# Autodesk Inventor assembly: playwood
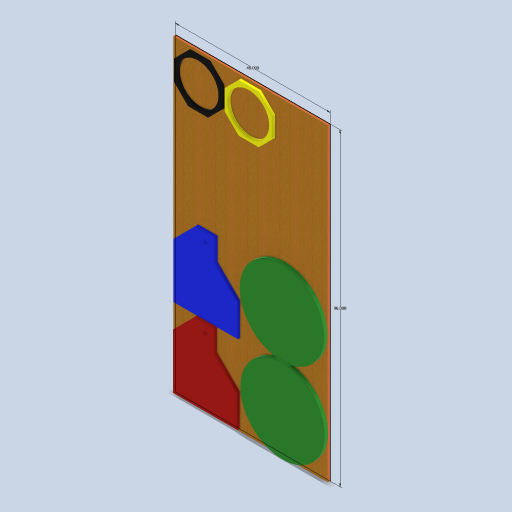
[picture p0: Inventor's stored thumbnail of the model, 512x512]
Saved by Autodesk Inventor 2023 (Build 270158000, 158)
## iProperties
Created: 2022-10-13
Part Number: playwood
Document SubType Name: Assembly
Designer: Nathan
Author: Nathan
## Documents named in this file (5)
- C:\Users\Nathan\Desktop\Senior Project\Schematics\playwood.iam
- C:\Users\Nathan\Desktop\Senior Project\Schematics\4x8plywood.ipt
- C:\Users\Nathan\Desktop\Senior Project\Schematics\base side.ipt
- C:\Users\Nathan\Desktop\Senior Project\Schematics\Bracket.ipt
- C:\Users\Nathan\Desktop\Senior Project\Schematics\base turntable.ipt
## Components (7 placed, 4 different names)
1. 4x8plywood:1 — Mate:1, Mate:2, Mate:3, Mate:4, Mate:5, Mate:6
2. base side:1 — Mate:6
3. base side:2 — Mate:5
4. Bracket:1 — Mate:1
5. Bracket:2 — Mate:2
6. base turntable:1 — Mate:4
7. base turntable:2 — Mate:3
## Relationships (6: Mate 6)
- Mate:1: 4x8plywood:1 ↔ Bracket:1
- Mate:2: 4x8plywood:1 ↔ Bracket:2
- Mate:3: 4x8plywood:1 ↔ base turntable:2
- Mate:4: 4x8plywood:1 ↔ base turntable:1
- Mate:5: 4x8plywood:1 ↔ base side:2
- Mate:6: 4x8plywood:1 ↔ base side:1
